# Autodesk Inventor assembly: plate
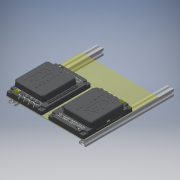
[picture p0: Inventor's stored thumbnail of the model, 180x180]
Saved by Autodesk Inventor 2019 (Build 230136000, 136)
## iProperties
Created: 2018-11-13
Part Number: plate
Document SubType Name: Assembly
Designer: User
Author: User
## Documents named in this file (4)
- C:\Robotics\CAD\2018-19_CAD\plate.iam
- C:\Robotics\CAD\2017-18_CAD\theplate.ipt
- C:\Robotics\CAD\COTSParts\Bosch Extrusion\Bosch 20x20 10in.ipt
- C:\Robotics\CAD\COTSParts\Rev\REV-31-1153RevHub.ipt
## Components (5 placed, 3 different names)
1. theplate:1 — Mate:1, Flush:1, Flush:2, Mate:2, Flush:4, Mate:3, Mate:4, Mate:6, Mate:7, Mate:9, Mate:10
2. Bosch 20x20 10in:1 — Mate:2, Flush:3, Flush:4
3. Bosch 20x20 10in:2 — Mate:1, Flush:1, Flush:2, Flush:3
4. REV-31-1153RevHub:2 — Mate:3, Mate:4, Mate:6, Mate:9, Flush:5
5. REV-31-1153RevHub:3 — Mate:7, Mate:10, Flush:5
## Relationships (13: Mate 8, Flush 5)
- Mate:1: theplate:1 ↔ Bosch 20x20 10in:2
- Flush:1: theplate:1 ↔ Bosch 20x20 10in:2
- Flush:2 (7.62 mm): theplate:1 ↔ Bosch 20x20 10in:2
- Mate:2: theplate:1 ↔ Bosch 20x20 10in:1
- Flush:3: Bosch 20x20 10in:1 ↔ Bosch 20x20 10in:2
- Flush:4: theplate:1 ↔ Bosch 20x20 10in:1
- Mate:3: theplate:1 ↔ REV-31-1153RevHub:2
- Mate:4: theplate:1 ↔ REV-31-1153RevHub:2
- Mate:6: theplate:1 ↔ REV-31-1153RevHub:2
- Mate:7: theplate:1 ↔ REV-31-1153RevHub:3
- Mate:9: theplate:1 ↔ REV-31-1153RevHub:2
- Mate:10: theplate:1 ↔ REV-31-1153RevHub:3
- Flush:5: REV-31-1153RevHub:2 ↔ REV-31-1153RevHub:3
